# Autodesk Inventor assembly: circular_stamp
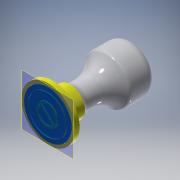
[picture p0: Inventor's stored thumbnail of the model, 180x180]
Saved by Autodesk Inventor 2019 (Build 230136000, 136)
## iProperties
Created: 2019-02-20
Part Number: circular_stamp
Document SubType Name: Assembly
Designer: jmc
Author: jmc
## Documents named in this file (4)
- C:\Users\l0086\Desktop\Models\Stamp\circular_stamp.iam
- C:\Users\l0086\Desktop\Models\Stamp\holder.ipt
- C:\Users\l0086\Desktop\Models\Stamp\holder_nut_circular.ipt
- C:\Users\l0086\Desktop\Models\Stamp\stamp_circular_hand.ipt
## Components (3 placed, 3 different names)
1. holder:1 — Rigid:2
2. holder_nut_circular:1 — Rigid:1, Rigid:2
3. stamp_circular_hand:1 — Rigid:1
## Relationships (2: WeldJoint 2)
- Rigid:1 [WeldJoint]: holder_nut_circular:1 ↔ stamp_circular_hand:1
- Rigid:2 [WeldJoint]: holder:1 ↔ holder_nut_circular:1
